# Autodesk Inventor assembly: 40TShaft
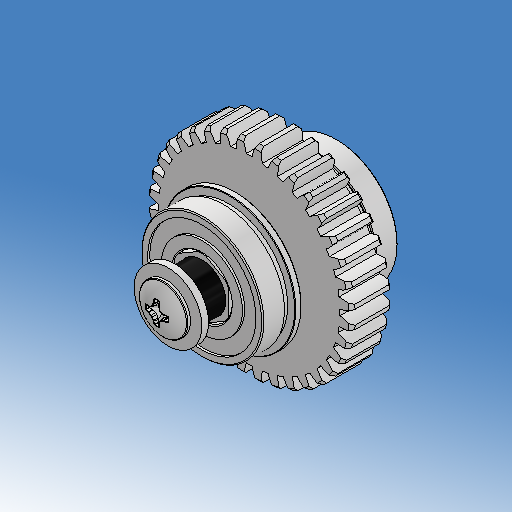
[picture p0: Inventor's stored thumbnail of the model, 512x512]
Saved by Autodesk Inventor 2025 (Build 290162000, 162)
## iProperties
Created: 2024-06-12
Part Number: 40TShaft
Document SubType Name: Assembly
Designer: seene
Author: seene
## Documents named in this file (8)
- C:\Users\seene\OneDrive\SBRT\Robocup Rescue\Drive\v1\36ShortShaft.iam
- C:\Users\seene\OneDrive\SBRT\Robocup Rescue\Drive\v1\REV-21-1916.ipt
- C:\Users\seene\OneDrive\SBRT\Robocup Rescue\Drive\v1\ShortRoundHexShaft.ipt
- C:\Users\seene\OneDrive\SBRT\Robocup Rescue\Drive\v1\Gears\am-4709 36T 20DP 500hex 375 FW.ipt
- C:\Users\seene\OneDrive\SBRT\Robocup Rescue\Drive\v1\2879T1_High-Load Oil-Embedded 863 Bronze Thrust Bearing.ipt
- C:\Users\seene\OneDrive\SBRT\Robocup Rescue\Drive\v1\91770A830_Extra-Wide Truss Head Phillips Screws.ipt
- C:\Users\seene\OneDrive\SBRT\Robocup Rescue\Drive\v1\HexBearingDrivePlateSapcer.ipt
- C:\Users\seene\OneDrive\SBRT\Robocup Rescue\Drive\v1\am-3948-063 500H x 063IN Spacer.ipt
## Components (11 placed, 7 different names)
1. REV-21-1916:1 — Mate:3, Mate:5, Flush:1, Mate:6, Mate:16, Mate:22
2. REV-21-1916:2 — Mate:3
3. ShortRoundHexShaft:1 — Mate:5, Flush:1, Mate:14, Mate:15, Mate:17
4. am-4709 36T 20DP 500hex 375 FW:1 — Mate:6, Mate:19, Mate:20, Mate:21, Mate:22
5. 2879T1_High-Load Oil-Embedded 863 Bronze Thrust Bearing:1 — Mate:7, Mate:8, Mate:9, Mate:12, Mate:13
6. 91770A830_Extra-Wide Truss Head Phillips Screws:1 — Mate:9, Mate:12, Mate:13
7. HexBearingDrivePlateSapcer:1 — Mate:7, Mate:8, Mate:14, Mate:15
8. 2879T1_High-Load Oil-Embedded 863 Bronze Thrust Bearing:2 — Mate:10, Mate:11, Mate:16, Mate:17
9. 91770A830_Extra-Wide Truss Head Phillips Screws:2 — Mate:10, Mate:11
10. am-3948-063 500H x 063IN Spacer:1 — Mate:18, Mate:21
11. am-3948-063 500H x 063IN Spacer:2 — Mate:18, Mate:19, Mate:20
## Relationships (20: Mate 19, Flush 1)
- Mate:3 (-19.05 mm): REV-21-1916:1 ↔ REV-21-1916:2
- Mate:5: REV-21-1916:1 ↔ ShortRoundHexShaft:1
- Flush:1: REV-21-1916:1 ↔ ShortRoundHexShaft:1
- Mate:6 (1.5875 mm): REV-21-1916:1 ↔ am-4709 36T 20DP 500hex 375 FW:1
- Mate:7: 2879T1_High-Load Oil-Embedded 863 Bronze Thrust Bearing:1 ↔ HexBearingDrivePlateSapcer:1
- Mate:8: 2879T1_High-Load Oil-Embedded 863 Bronze Thrust Bearing:1 ↔ HexBearingDrivePlateSapcer:1
- Mate:9: 2879T1_High-Load Oil-Embedded 863 Bronze Thrust Bearing:1 ↔ 91770A830_Extra-Wide Truss Head Phillips Screws:1
- Mate:10: 2879T1_High-Load Oil-Embedded 863 Bronze Thrust Bearing:2 ↔ 91770A830_Extra-Wide Truss Head Phillips Screws:2
- Mate:11: 2879T1_High-Load Oil-Embedded 863 Bronze Thrust Bearing:2 ↔ 91770A830_Extra-Wide Truss Head Phillips Screws:2
- Mate:12: 2879T1_High-Load Oil-Embedded 863 Bronze Thrust Bearing:1 ↔ 91770A830_Extra-Wide Truss Head Phillips Screws:1
- Mate:13: 2879T1_High-Load Oil-Embedded 863 Bronze Thrust Bearing:1 ↔ 91770A830_Extra-Wide Truss Head Phillips Screws:1
- Mate:14: ShortRoundHexShaft:1 ↔ HexBearingDrivePlateSapcer:1
- Mate:15: ShortRoundHexShaft:1 ↔ HexBearingDrivePlateSapcer:1
- Mate:16: REV-21-1916:1 ↔ 2879T1_High-Load Oil-Embedded 863 Bronze Thrust Bearing:2
- Mate:17: ShortRoundHexShaft:1 ↔ 2879T1_High-Load Oil-Embedded 863 Bronze Thrust Bearing:2
- Mate:18: am-3948-063 500H x 063IN Spacer:1 ↔ am-3948-063 500H x 063IN Spacer:2
- Mate:19: am-4709 36T 20DP 500hex 375 FW:1 ↔ am-3948-063 500H x 063IN Spacer:2
- Mate:20: am-4709 36T 20DP 500hex 375 FW:1 ↔ am-3948-063 500H x 063IN Spacer:2
- Mate:21: am-4709 36T 20DP 500hex 375 FW:1 ↔ am-3948-063 500H x 063IN Spacer:1
- Mate:22: REV-21-1916:1 ↔ am-4709 36T 20DP 500hex 375 FW:1
## Named parameters: Finish1_Area = 12.8877
note: some values were not read from the file. Shown as the stored number, unit unknown: "Finish1_Area".
